# Autodesk Inventor assembly: Normal Wheel Assembly
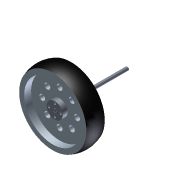
[picture p0: Inventor's stored thumbnail of the model, 180x180]
Saved by Autodesk Inventor 2015 SP1 (Build 190203100, 203)
## iProperties
Created: 2015-01-22
Part Number: Normal Wheel Assembly
Document SubType Name: Assembly
Designer: rihoobler
Author: rihoobler
## Documents named in this file (7)
- C:\Users\datenney\Documents\GitHub\CAD\SerenityMk.2\Normal Wheel Assembly.iam
- C:\Users\rihoobler\Documents\Inventor\tetrix_739055_2012.ipt
- C:\Users\datenney\Documents\GitHub\CAD\SerenityMk.2\Imported Components\tetrix_739088_2012\tetrix_739088_2012.ipt
- C:\Users\datenney\Documents\GitHub\CAD\SerenityMk.2\Imported Components\tetrix_739172_2012\tetrix_739172_2012.iam
- C:\Users\datenney\Documents\GitHub\CAD\SerenityMk.2\Imported Components\tetrix_739165_2012\tetrix_739165_2012.ipt
- C:\Users\datenney\Documents\GitHub\CAD\SerenityMk.2\Imported Components\tetrix_739090_2012\tetrix_739090_2012.ipt
- C:\Users\datenney\Documents\GitHub\CAD\SerenityMk.2\Imported Components\tetrix_739100_2012\tetrix_739100_2012.ipt
## Components (6 placed, 6 different names)
1. tetrix_739055_2012:1 — Insert:1, Mate:2, Insert:2
2. tetrix_739088_2012:1 — Mate:2, Flush:1
3. tetrix_739172_2012:2 [sub-assembly] — Insert:1, Flush:1
4. tetrix_739165_2012:1 — Insert:3, Insert:4
5. tetrix_739090_2012:1 — Insert:2, Insert:3
6. tetrix_739100_2012:1 — Insert:4
## Relationships (6: Insert 4, Mate 1, Flush 1)
- Insert:1: tetrix_739055_2012:1 ↔ tetrix_739172_2012:2
- Mate:2: tetrix_739055_2012:1 ↔ tetrix_739088_2012:1
- Flush:1: tetrix_739088_2012:1 ↔ tetrix_739172_2012:2
- Insert:2: tetrix_739055_2012:1 ↔ tetrix_739090_2012:1
- Insert:3: tetrix_739165_2012:1 ↔ tetrix_739090_2012:1
- Insert:4: tetrix_739165_2012:1 ↔ tetrix_739100_2012:1
